# Autodesk Inventor assembly: RCUAssy
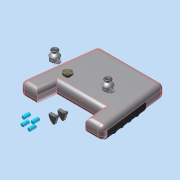
[picture p0: Inventor's stored thumbnail of the model, 180x180]
Saved by Autodesk Inventor 2011 SP1 (Build 150282100, 282)
## iProperties
Created: 2011-08-16
Part Number: RCUAssy
Document SubType Name: Assembly
Designer: dgitz
Author: dgitz
## Documents named in this file (8)
- C:\Dropbox\ICARUS\Remote Control Unit (RCU)\RCU v2\Design\RCUv2-4\RCUAssy.iam
- C:\Dropbox\ICARUS\Remote Control Unit (RCU)\RCU v2\Design\RCUv2-4\RUCBase.ipt
- C:\Dropbox\ICARUS\Remote Control Unit (RCU)\RCU v2\Design\RCUv2-4\Grip.ipt
- C:\Dropbox\ICARUS\Remote Control Unit (RCU)\RCU v2\Design\Library\XBox360DirectionalPad.ipt
- C:\Dropbox\ICARUS\Remote Control Unit (RCU)\RCU v2\Design\Library\Xbox360Button.ipt
- C:\Dropbox\ICARUS\Remote Control Unit (RCU)\RCU v2\Design\Library\Trigger.ipt
- C:\Dropbox\ICARUS\Remote Control Unit (RCU)\RCU v2\Design\Imported Components\User Library-Joystick_Asm_Left\Assembly2.iam
- C:\Dropbox\ICARUS\Remote Control Unit (RCU)\RCU v2\Design\Library\XBeeAntennaAssy.iam
## Components (13 placed, 7 different names)
1. RUCBase:1 — Mate:1, Mate:2, Mate:3, Flush:1, Flush:2, Mate:4, Mate:5, Mate:6, Mate:7, Mate:8, Mate:9, Mate:13, Mate:14, Mate:16
2. Grip:1 — Mate:1, Mate:2, Mate:3
3. Grip:2 — Mate:4, Mate:5, Mate:6
4. XBox360DirectionalPad:1 — Mate:7
5. Xbox360Button:1 — Flush:4, Flush:5, Mate:11, Mate:12
6. Xbox360Button:2 — Flush:5, Mate:12
7. Xbox360Button:3 — Flush:3, Mate:10, Mate:13
8. Xbox360Button:4 — Flush:3, Flush:4, Mate:10, Mate:11
9. Assembly2:1 [sub-assembly] — Mate:9
10. Assembly2:2 [sub-assembly] — Mate:8
11. Trigger:1 — Insert:1, Angle:1, Mate:14, Mate:15
12. Trigger:2 — Insert:1, Angle:1
13. XBeeAntennaAssy:1 [sub-assembly] — Mate:16, Mate:17
## Relationships (24: Mate 17, Flush 5, Insert 1, Angle 1)
- Mate:1: RUCBase:1 ↔ Grip:1
- Mate:2: RUCBase:1 ↔ Grip:1
- Mate:3 (12.7 mm): RUCBase:1 ↔ Grip:1
- Flush:1: RUCBase:1
- Flush:2: RUCBase:1
- Mate:4: RUCBase:1 ↔ Grip:2
- Mate:5: RUCBase:1 ↔ Grip:2
- Mate:6 (12.7 mm): RUCBase:1 ↔ Grip:2
- Mate:7: RUCBase:1 ↔ XBox360DirectionalPad:1
- Mate:8 (-3.175 mm): RUCBase:1 ↔ Assembly2:2
- Mate:9 (-3.175 mm): RUCBase:1 ↔ Assembly2:1
- Flush:3: Xbox360Button:3 ↔ Xbox360Button:4
- Flush:4: Xbox360Button:1 ↔ Xbox360Button:4
- Flush:5: Xbox360Button:1 ↔ Xbox360Button:2
- Mate:10 (12.7 mm): Xbox360Button:3 ↔ Xbox360Button:4
- Mate:11 (12.7 mm): Xbox360Button:1 ↔ Xbox360Button:4
- Mate:12 (12.7 mm): Xbox360Button:1 ↔ Xbox360Button:2
- Mate:13 (-12.7 mm): RUCBase:1 ↔ Xbox360Button:3
- Insert:1 (101.6 mm): Trigger:1 ↔ Trigger:2
- Angle:1 (0 deg): Trigger:1 ↔ Trigger:2
- Mate:14 (-6.35 mm): RUCBase:1 ↔ Trigger:1
- Mate:15: Trigger:1
- Mate:16: RUCBase:1 ↔ XBeeAntennaAssy:1
- Mate:17 (50.8 mm): XBeeAntennaAssy:1
